# Autodesk Inventor assembly: lifting mechanism
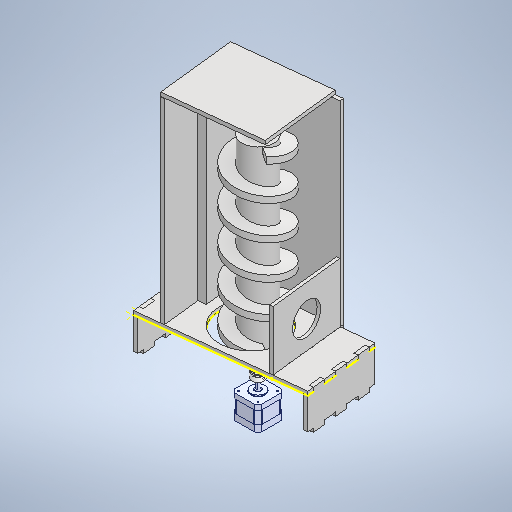
[picture p0: Inventor's stored thumbnail of the model, 512x512]
Saved by Autodesk Inventor 2025.3 (Build 293356000, 356)
## iProperties
Created: 2026-04-14
Part Number: lifting mechanism
Document SubType Name: Assembly
Designer: ziada
Author: ziada
## Documents named in this file (11)
- C:\Users\kamal\OneDrive\Desktop\Personal\semester 4\Basics of Mechatronics\Full Assembly\lifting mechanism.iam
- C:\Users\kamal\OneDrive\Desktop\Personal\semester 4\Basics of Mechatronics\Full Assembly\NEMA17 Model STEP\NEMA17 Model STEP\NEMA17 Model STEP.iam
- C:\Users\kamal\OneDrive\Desktop\Personal\semester 4\Basics of Mechatronics\Full Assembly\Flexible Shaft Coupler 5x8mm\Flexible Shaft Coupler 5x8mm\Flexible Shaft Coupler 5x8mm.ipt
- C:\Users\kamal\OneDrive\Desktop\Personal\semester 4\Basics of Mechatronics\Full Assembly\Archimedes Screw V2.ipt
- C:\Users\kamal\OneDrive\Desktop\Personal\semester 4\Basics of Mechatronics\Full Assembly\Insert.ipt
- C:\Users\kamal\OneDrive\Desktop\Personal\semester 4\Basics of Mechatronics\Full Assembly\Wall.ipt
- C:\Users\kamal\OneDrive\Desktop\Personal\semester 4\Basics of Mechatronics\Full Assembly\Top.ipt
- C:\Users\kamal\OneDrive\Desktop\Personal\semester 4\Basics of Mechatronics\Full Assembly\Wall2.ipt
- C:\Users\kamal\OneDrive\Desktop\Personal\semester 4\Basics of Mechatronics\Full Assembly\Exit.ipt
- C:\Users\kamal\OneDrive\Desktop\Personal\semester 4\Basics of Mechatronics\Full Assembly\Base Connection.ipt
- C:\Users\kamal\OneDrive\Desktop\Personal\semester 4\Basics of Mechatronics\Full Assembly\Base lif.ipt
## Components (11 placed, 10 different names)
1. NEMA17 Model STEP:1 [sub-assembly] — Insert:1
2. Flexible Shaft Coupler 5x8mm:1 — Insert:1, Insert:2
3. Archimedes Screw V2:1 — Insert:2
4. Top:1 — Mate:35, Mate:36
5. Wall:1 — Mate:27, Mate:30, Mate:31, Mate:32
6. Wall2:1 — Mate:31, Mate:32, Mate:35
7. Exit:1 — Mate:33, Mate:34, Mate:36
8. Insert:1 — Mate:25, Mate:26
9. Base lif:1 — Mate:25, Mate:26, Mate:27, Mate:30, Mate:33, Mate:34, Mate:37, Mate:38, Mate:39, Mate:40
10. Base Connection:1 — Mate:37, Mate:38
11. Base Connection:2 — Mate:39, Mate:40
## Relationships (16: Mate 14, Insert 2)
- Insert:1 (-5 mm): NEMA17 Model STEP:1 ↔ Flexible Shaft Coupler 5x8mm:1
- Insert:2 (-5 mm): Flexible Shaft Coupler 5x8mm:1 ↔ Archimedes Screw V2:1
- Mate:25: Insert:1 ↔ Base lif:1
- Mate:26: Insert:1 ↔ Base lif:1
- Mate:27: Wall:1 ↔ Base lif:1
- Mate:30: Wall:1 ↔ Base lif:1
- Mate:31: Wall:1 ↔ Wall2:1
- Mate:32: Wall:1 ↔ Wall2:1
- Mate:33: Exit:1 ↔ Base lif:1
- Mate:34: Exit:1 ↔ Base lif:1
- Mate:35: Top:1 ↔ Wall2:1
- Mate:36: Top:1 ↔ Exit:1
- Mate:37: Base lif:1 ↔ Base Connection:1
- Mate:38: Base lif:1 ↔ Base Connection:1
- Mate:39: Base lif:1 ↔ Base Connection:2
- Mate:40: Base lif:1 ↔ Base Connection:2
